# Autodesk Inventor assembly: base_assambly
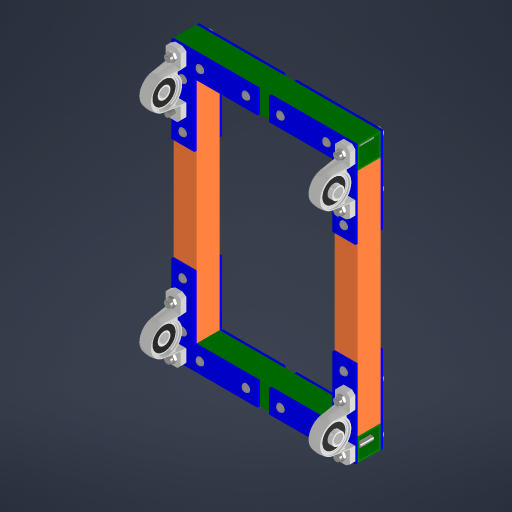
[picture p0: Inventor's stored thumbnail of the model, 512x512]
Saved by Autodesk Inventor 2024 (Build 280153000, 153)
## iProperties
Created: 2023-09-25
Part Number: base_assambly
Document SubType Name: Assembly
Designer: user
Author: user
## Documents named in this file (8)
- D:\Docs\Robot\3d_v2\base\base_assambly.iam
- D:\Docs\Robot\3d_v2\base\fb_axis.ipt
- D:\Docs\Robot\3d_v2\base\side_axis.ipt
- D:\Docs\Robot\3d_v2\default_components\mounting_bracket.ipt
- D:\Docs\Robot\3d_v2\default_components\fasteners\DIN 660 - B 4 x 8 x 1,9.ipt
- D:\Docs\Robot\3d_v2\default_components\KP08.iam
- C:\Users\user\Documents\Inventor\Content Center Files\R2024\ru-RU\ISO 4762(1)\DIN EN ISO 4762 - M4 x 35.ipt
- C:\Users\user\Documents\Inventor\Content Center Files\R2024\ru-RU\DIN 985\DIN 985 - M4.ipt
## Components (63 placed, 7 different names)
1. fb_axis:1 — Совмещение:6, Заподлицо:5, Заподлицо:6, Совмещение:10, Заподлицо:7, Совмещение:12, Совмещение:19, Вставка:19, Вставка:24, Симметрия:1
2. side_axis:1 — Совмещение:1, Совмещение:2, Совмещение:3, Совмещение:4, Заподлицо:1, Заподлицо:2, Заподлицо:13, Совмещение:14, Совмещение:16, Вставка:21, Вставка:23
3. fb_axis:2 — Совмещение:4, Заподлицо:1, Заподлицо:2, Заподлицо:3, Заподлицо:4, Совмещение:5, Заподлицо:10, Совмещение:21, Вставка:22, Вставка:25, Симметрия:1
4. side_axis:2 — Заподлицо:3, Заподлицо:4, Совмещение:5, Совмещение:6, Заподлицо:5, Заподлицо:6, Совмещение:8, Заподлицо:9, Совмещение:18, Вставка:20, Вставка:26
5. KP08:4 [sub-assembly] — Вставка:27, Вставка:28, Вставка:66, Вставка:67
6. KP08:3 [sub-assembly] — Вставка:33, Вставка:34, Вставка:68, Вставка:69
7. KP08:2 [sub-assembly] — Вставка:29, Вставка:30, Вставка:56, Вставка:65
8. KP08:1 [sub-assembly] — Вставка:31, Вставка:32, Вставка:64
9. mounting_bracket:11 — Вставка:23, Вставка:24, Вставка:51, Вставка:52, Вставка:53, Вставка:54, Вставка:60, Вставка:61
10. mounting_bracket:12 — Вставка:25, Вставка:26, Вставка:47, Вставка:48, Вставка:49, Вставка:50, Вставка:55, Вставка:57
11. mounting_bracket:10 — Вставка:21, Вставка:22, Вставка:31, Вставка:32, Вставка:39, Вставка:40, Вставка:41, Вставка:42
12. mounting_bracket:9 — Вставка:19, Вставка:20, Вставка:27, Вставка:28, Вставка:35, Вставка:36, Вставка:37, Вставка:38
13. mounting_bracket:6 — Совмещение:12, Совмещение:18, Совмещение:19, Вставка:3, Вставка:4, Вставка:5, Вставка:6, Вставка:58, Вставка:59
14. mounting_bracket:4 — Совмещение:8, Заподлицо:9, Заподлицо:10, Вставка:29, Вставка:30, Вставка:43, Вставка:44, Вставка:45, Вставка:46
15. mounting_bracket:3 — Совмещение:10, Заподлицо:7, Заподлицо:13, Совмещение:25, Совмещение:26, Совмещение:27, Совмещение:28, Вставка:33, Вставка:34
16. mounting_bracket:8 — Совмещение:14, Совмещение:16, Совмещение:21, Вставка:15, Вставка:16, Вставка:17, Вставка:18, Вставка:62, Вставка:63
17. DIN 660 - B 4 x 8 x 1,9:63 — Вставка:51
18. DIN 660 - B 4 x 8 x 1,9:60 — Вставка:50
19. DIN 660 - B 4 x 8 x 1,9:53 — Вставка:49
20. DIN 660 - B 4 x 8 x 1,9:51 — Вставка:47
21. DIN 660 - B 4 x 8 x 1,9:52 — Вставка:48
22. DIN 660 - B 4 x 8 x 1,9:56 — Вставка:54
23. DIN 660 - B 4 x 8 x 1,9:57 — Вставка:53
24. DIN 660 - B 4 x 8 x 1,9:62 — Вставка:52
25. DIN 660 - B 4 x 8 x 1,9:39 — Вставка:38
26. DIN 660 - B 4 x 8 x 1,9:40 — Вставка:36
27. DIN 660 - B 4 x 8 x 1,9:42 — Вставка:35
28. DIN 660 - B 4 x 8 x 1,9:41 — Вставка:37
29. DIN 660 - B 4 x 8 x 1,9:43 — Вставка:39
30. DIN 660 - B 4 x 8 x 1,9:45 — Вставка:43
31. DIN 660 - B 4 x 8 x 1,9:44 — Вставка:44
32. DIN 660 - B 4 x 8 x 1,9:46 — Вставка:42
33. DIN 660 - B 4 x 8 x 1,9:47 — Вставка:40
34. DIN 660 - B 4 x 8 x 1,9:48 — Вставка:41
35. DIN 660 - B 4 x 8 x 1,9:49 — Вставка:45
36. DIN 660 - B 4 x 8 x 1,9:50 — Вставка:46
37. DIN 660 - B 4 x 8 x 1,9:10 — Совмещение:28
38. DIN 660 - B 4 x 8 x 1,9:5 — Совмещение:25
39. DIN 660 - B 4 x 8 x 1,9:29 — Вставка:5
40. DIN 660 - B 4 x 8 x 1,9:27 — Вставка:6
41. DIN 660 - B 4 x 8 x 1,9:13 — Совмещение:26
42. DIN 660 - B 4 x 8 x 1,9:12 — Совмещение:27
43. DIN 660 - B 4 x 8 x 1,9:21 — Вставка:4
44. DIN 660 - B 4 x 8 x 1,9:24 — Вставка:15
45. DIN 660 - B 4 x 8 x 1,9:28 — Вставка:3
46. DIN 660 - B 4 x 8 x 1,9:34 — Вставка:17
47. DIN 660 - B 4 x 8 x 1,9:38 — Вставка:16
48. DIN 660 - B 4 x 8 x 1,9:35 — Вставка:18
49. DIN EN ISO 4762 M4 x 35:8 — Вставка:61
50. DIN EN ISO 4762 M4 x 35:7 — Вставка:62
51. DIN EN ISO 4762 M4 x 35:6 — Вставка:63
52. DIN EN ISO 4762 M4 x 35:5 — Вставка:60
53. DIN EN ISO 4762 M4 x 35:4 — Вставка:59
54. DIN EN ISO 4762 M4 x 35:3 — Вставка:58
55. DIN EN ISO 4762 M4 x 35:2 — Вставка:57
56. DIN EN ISO 4762 M4 x 35:1 — Вставка:55
57. DIN 985 - заменено на DIN EN ISO 10511 M4:14 — Вставка:65
58. DIN 985 - заменено на DIN EN ISO 10511 M4:13 — Вставка:64
59. DIN 985 - заменено на DIN EN ISO 10511 M4:10 — Вставка:69
60. DIN 985 - заменено на DIN EN ISO 10511 M4:6 — Вставка:68
61. DIN 985 - заменено на DIN EN ISO 10511 M4:2 — Вставка:66
62. DIN 985 - заменено на DIN EN ISO 10511 M4:7 — Вставка:67
63. DIN 985 - заменено на DIN EN ISO 10511 M4:1 — Вставка:56
## Relationships (88: Insert 59, Mate 18, Flush 10, Symmetry 1)
- Совмещение:1 [Mate]: side_axis:1
- Совмещение:2 [Mate]: side_axis:1
- Совмещение:3 [Mate]: side_axis:1
- Совмещение:4 [Mate]: side_axis:1 ↔ fb_axis:2
- Заподлицо:1 [Flush]: side_axis:1 ↔ fb_axis:2
- Заподлицо:2 [Flush]: side_axis:1 ↔ fb_axis:2
- Заподлицо:3 [Flush]: fb_axis:2 ↔ side_axis:2
- Заподлицо:4 [Flush]: fb_axis:2 ↔ side_axis:2
- Совмещение:5 [Mate]: fb_axis:2 ↔ side_axis:2
- Совмещение:6 [Mate]: fb_axis:1 ↔ side_axis:2
- Заподлицо:5 [Flush]: fb_axis:1 ↔ side_axis:2
- Заподлицо:6 [Flush]: fb_axis:1 ↔ side_axis:2
- Совмещение:8 [Mate]: side_axis:2 ↔ mounting_bracket:4
- Совмещение:10 [Mate]: fb_axis:1 ↔ mounting_bracket:3
- Заподлицо:7 [Flush]: fb_axis:1 ↔ mounting_bracket:3
- Заподлицо:9 [Flush]: side_axis:2 ↔ mounting_bracket:4
- Заподлицо:10 [Flush]: fb_axis:2 ↔ mounting_bracket:4
- Заподлицо:13 [Flush]: side_axis:1 ↔ mounting_bracket:3
- Совмещение:12 [Mate]: fb_axis:1 ↔ mounting_bracket:6
- Совмещение:14 [Mate]: side_axis:1 ↔ mounting_bracket:8
- Совмещение:16 [Mate]: side_axis:1 ↔ mounting_bracket:8
- Совмещение:18 [Mate]: side_axis:2 ↔ mounting_bracket:6
- Совмещение:19 [Mate]: fb_axis:1 ↔ mounting_bracket:6
- Совмещение:21 [Mate]: fb_axis:2 ↔ mounting_bracket:8
- Совмещение:25 [Mate]: mounting_bracket:3 ↔ DIN 660 - B 4 x 8 x 1,9:5
- Совмещение:26 [Mate]: mounting_bracket:3 ↔ DIN 660 - B 4 x 8 x 1,9:13
- Совмещение:27 [Mate]: mounting_bracket:3 ↔ DIN 660 - B 4 x 8 x 1,9:12
- Совмещение:28 [Mate]: mounting_bracket:3 ↔ DIN 660 - B 4 x 8 x 1,9:10
- Вставка:3 [Insert]: mounting_bracket:6 ↔ DIN 660 - B 4 x 8 x 1,9:28
- Вставка:4 [Insert]: mounting_bracket:6 ↔ DIN 660 - B 4 x 8 x 1,9:21
- Вставка:5 [Insert]: mounting_bracket:6 ↔ DIN 660 - B 4 x 8 x 1,9:29
- Вставка:6 [Insert]: mounting_bracket:6 ↔ DIN 660 - B 4 x 8 x 1,9:27
- Вставка:15 [Insert]: mounting_bracket:8 ↔ DIN 660 - B 4 x 8 x 1,9:24
- Вставка:16 [Insert]: mounting_bracket:8 ↔ DIN 660 - B 4 x 8 x 1,9:38
- Вставка:17 [Insert]: mounting_bracket:8 ↔ DIN 660 - B 4 x 8 x 1,9:34
- Вставка:18 [Insert]: mounting_bracket:8 ↔ DIN 660 - B 4 x 8 x 1,9:35
- Вставка:19 [Insert]: fb_axis:1 ↔ mounting_bracket:9
- Вставка:20 [Insert]: side_axis:2 ↔ mounting_bracket:9
- Вставка:21 [Insert]: side_axis:1 ↔ mounting_bracket:10
- Вставка:22 [Insert]: fb_axis:2 ↔ mounting_bracket:10
- Вставка:23 [Insert]: side_axis:1 ↔ mounting_bracket:11
- Вставка:24 [Insert]: fb_axis:1 ↔ mounting_bracket:11
- Вставка:25 [Insert]: fb_axis:2 ↔ mounting_bracket:12
- Вставка:26 [Insert]: side_axis:2 ↔ mounting_bracket:12
- Вставка:27 [Insert]: KP08:4 ↔ mounting_bracket:9
- Вставка:28 [Insert]: KP08:4 ↔ mounting_bracket:9
- Вставка:29 [Insert]: KP08:2 ↔ mounting_bracket:4
- Вставка:30 [Insert]: KP08:2 ↔ mounting_bracket:4
- Вставка:31 [Insert]: KP08:1 ↔ mounting_bracket:10
- Вставка:32 [Insert]: KP08:1 ↔ mounting_bracket:10
- Вставка:33 [Insert]: KP08:3 ↔ mounting_bracket:3
- Вставка:34 [Insert]: KP08:3 ↔ mounting_bracket:3
- Вставка:35 [Insert]: mounting_bracket:9 ↔ DIN 660 - B 4 x 8 x 1,9:42
- Вставка:36 [Insert]: mounting_bracket:9 ↔ DIN 660 - B 4 x 8 x 1,9:40
- Вставка:37 [Insert]: mounting_bracket:9 ↔ DIN 660 - B 4 x 8 x 1,9:41
- Вставка:38 [Insert]: mounting_bracket:9 ↔ DIN 660 - B 4 x 8 x 1,9:39
- Вставка:39 [Insert]: mounting_bracket:10 ↔ DIN 660 - B 4 x 8 x 1,9:43
- Вставка:40 [Insert]: mounting_bracket:10 ↔ DIN 660 - B 4 x 8 x 1,9:47
- Вставка:41 [Insert]: mounting_bracket:10 ↔ DIN 660 - B 4 x 8 x 1,9:48
- Вставка:42 [Insert]: mounting_bracket:10 ↔ DIN 660 - B 4 x 8 x 1,9:46
- Вставка:43 [Insert]: mounting_bracket:4 ↔ DIN 660 - B 4 x 8 x 1,9:45
- Вставка:44 [Insert]: mounting_bracket:4 ↔ DIN 660 - B 4 x 8 x 1,9:44
- Вставка:45 [Insert]: mounting_bracket:4 ↔ DIN 660 - B 4 x 8 x 1,9:49
- Вставка:46 [Insert]: mounting_bracket:4 ↔ DIN 660 - B 4 x 8 x 1,9:50
- Вставка:47 [Insert]: mounting_bracket:12 ↔ DIN 660 - B 4 x 8 x 1,9:51
- Вставка:48 [Insert]: mounting_bracket:12 ↔ DIN 660 - B 4 x 8 x 1,9:52
- Вставка:49 [Insert]: mounting_bracket:12 ↔ DIN 660 - B 4 x 8 x 1,9:53
- Вставка:50 [Insert]: mounting_bracket:12 ↔ DIN 660 - B 4 x 8 x 1,9:60
- Вставка:51 [Insert]: mounting_bracket:11 ↔ DIN 660 - B 4 x 8 x 1,9:63
- Вставка:52 [Insert]: mounting_bracket:11 ↔ DIN 660 - B 4 x 8 x 1,9:62
- Вставка:53 [Insert]: mounting_bracket:11 ↔ DIN 660 - B 4 x 8 x 1,9:57
- Вставка:54 [Insert]: mounting_bracket:11 ↔ DIN 660 - B 4 x 8 x 1,9:56
- Вставка:55 [Insert]: mounting_bracket:12 ↔ DIN EN ISO 4762 M4 x 35:1
- Вставка:56 [Insert]: KP08:2 ↔ DIN 985 - заменено на DIN EN ISO 10511 M4:1
- Вставка:57 [Insert]: mounting_bracket:12 ↔ DIN EN ISO 4762 M4 x 35:2
- Вставка:58 [Insert]: mounting_bracket:6 ↔ DIN EN ISO 4762 M4 x 35:3
- Вставка:59 [Insert]: mounting_bracket:6 ↔ DIN EN ISO 4762 M4 x 35:4
- Вставка:60 [Insert]: mounting_bracket:11 ↔ DIN EN ISO 4762 M4 x 35:5
- Вставка:61 [Insert]: mounting_bracket:11 ↔ DIN EN ISO 4762 M4 x 35:8
- Вставка:62 [Insert]: mounting_bracket:8 ↔ DIN EN ISO 4762 M4 x 35:7
- Вставка:63 [Insert]: mounting_bracket:8 ↔ DIN EN ISO 4762 M4 x 35:6
- Вставка:64 [Insert]: KP08:1 ↔ DIN 985 - заменено на DIN EN ISO 10511 M4:13
- Вставка:65 [Insert]: KP08:2 ↔ DIN 985 - заменено на DIN EN ISO 10511 M4:14
- Вставка:66 [Insert]: KP08:4 ↔ DIN 985 - заменено на DIN EN ISO 10511 M4:2
- Вставка:67 [Insert]: KP08:4 ↔ DIN 985 - заменено на DIN EN ISO 10511 M4:7
- Вставка:68 [Insert]: KP08:3 ↔ DIN 985 - заменено на DIN EN ISO 10511 M4:6
- Вставка:69 [Insert]: KP08:3 ↔ DIN 985 - заменено на DIN EN ISO 10511 M4:10
- Симметрия:1 [Symmetry]: fb_axis:1 ↔ fb_axis:2
